# Autodesk Inventor assembly: PP_T0.75_01
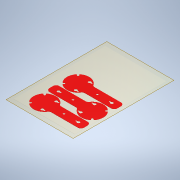
[picture p0: Inventor's stored thumbnail of the model, 180x180]
Saved by Autodesk Inventor 2020 (Build 240168000, 168)
## iProperties
Created: 2021-08-27
Part Number: PP_T0.75_01
Document SubType Name: Assembly
Designer: Masato
Author: Masato
## Documents named in this file (3)
- C:\Users\marin\Documents\0325 git clone\SUSTAINA-OP\Cam\PP_T0.75_01.iam
- C:\Users\marin\Documents\0325 git clone\SUSTAINA-OP\Cam\DisposableBoard.ipt
- C:\Users\marin\Documents\0420 git clone\SUSTAINA-OP\UpperBody\Arm\ForeArm_outside_cloth.ipt
## Components (4 placed, 2 different names)
1. DisposableBoard:1 — メイト:2, メイト:1, フラッシュ:1, フラッシュ:2, フラッシュ:3, 正接:1, 角度:1, 正接:2, メイト:6, フラッシュ:4
2. ForeArm_outside_cloth:1 — メイト:5, 角度:1, 正接:2, 正接:3, 正接:4
3. ForeArm_outside_cloth:2 — メイト:4, フラッシュ:3, 正接:1, 正接:3
4. ForeArm_outside_cloth:3 — メイト:6, フラッシュ:4, 正接:4
## Relationships (14: Mate 5, Flush 4, Tangent 4, Angle 1)
- メイト:2 [Mate]: DisposableBoard:1
- メイト:1 [Mate]: DisposableBoard:1
- フラッシュ:1 [Flush]: DisposableBoard:1
- フラッシュ:2 [Flush]: DisposableBoard:1
- メイト:4 [Mate]: ForeArm_outside_cloth:2
- フラッシュ:3 [Flush] (3 mm): DisposableBoard:1 ↔ ForeArm_outside_cloth:2
- 正接:1 [Tangent] (3 mm): DisposableBoard:1 ↔ ForeArm_outside_cloth:2
- メイト:5 [Mate]: ForeArm_outside_cloth:1
- 角度:1 [Angle] (0 deg): DisposableBoard:1 ↔ ForeArm_outside_cloth:1
- 正接:2 [Tangent]: DisposableBoard:1 ↔ ForeArm_outside_cloth:1
- 正接:3 [Tangent] (2.5 mm): ForeArm_outside_cloth:1 ↔ ForeArm_outside_cloth:2
- メイト:6 [Mate]: DisposableBoard:1 ↔ ForeArm_outside_cloth:3
- フラッシュ:4 [Flush] (3 mm): DisposableBoard:1 ↔ ForeArm_outside_cloth:3
- 正接:4 [Tangent] (2.5 mm): ForeArm_outside_cloth:1 ↔ ForeArm_outside_cloth:3
